# Autodesk Inventor assembly: Clamping collar 1_4 Assembly
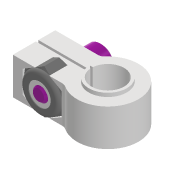
[picture p0: Inventor's stored thumbnail of the model, 180x180]
Saved by Autodesk Inventor 2020 (Build 240168000, 168)
## iProperties
Created: 2019-11-09
Part Number: Clamping collar 1_4 Assembly
Document SubType Name: Assembly
Designer: ball
Author: ball
## Documents named in this file (4)
- C:\FTC\FTC8863CAD\2019 Robot\Generic Parts\Clamping collar 1_4 Assembly.iam
- C:\FTC\FTC8863CAD\2019 Robot\Generic Parts\Clamping Collar 1_4.ipt
- C:\FTC\FTC8863CAD\StepLibraries\Nuts\6-32 NYLON-INSERT LOCKNUT.ipt
- C:\FTC\FTC8863CAD\StepLibraries\Screws\6-32x.375 SOCKET HEAD CAP SCREW.ipt
## Components (3 placed, 3 different names)
1. Clamping Collar 1_4:1 — Mate:1, Mate:2, Angle:1, Mate:3, Mate:4
2. 6-32 NYLON-INSERT LOCKNUT:1 — Mate:1, Mate:2, Angle:1
3. 6-32x.375 SOCKET HEAD CAP SCREW:1 — Mate:3, Mate:4
## Relationships (5: Mate 4, Angle 1)
- Mate:1: Clamping Collar 1_4:1 ↔ 6-32 NYLON-INSERT LOCKNUT:1
- Mate:2: Clamping Collar 1_4:1 ↔ 6-32 NYLON-INSERT LOCKNUT:1
- Angle:1 (0 deg): Clamping Collar 1_4:1 ↔ 6-32 NYLON-INSERT LOCKNUT:1
- Mate:3: Clamping Collar 1_4:1 ↔ 6-32x.375 SOCKET HEAD CAP SCREW:1
- Mate:4: Clamping Collar 1_4:1 ↔ 6-32x.375 SOCKET HEAD CAP SCREW:1
